# Autodesk Inventor assembly: OttosBreadboard_ASM
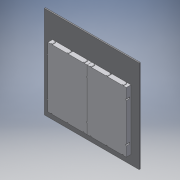
[picture p0: Inventor's stored thumbnail of the model, 180x180]
Saved by Autodesk Inventor 2016 (Build 200138000, 138)
## iProperties
Created: 2018-06-19
Part Number: OttosBreadboard_ASM
Document SubType Name: Assembly
Designer: suku
Author: suku
## Documents named in this file (3)
- I:\SukuWc\Otto's DIY\Core\Breadboard\OttosBreadboard_ASM.iam
- I:\SukuWc\Otto's DIY\Core\Breadboard\OttosBreadboard.ipt
- I:\SukuWc\Otto's DIY\Core\Breadboard\Frontpanel.ipt
## Components (3 placed, 2 different names)
1. OttosBreadboard:1 — Flush:1, Flush:2, Mate:1
2. OttosBreadboard:2 — Flush:1, Flush:2, Mate:1, Flush:3
3. Frontpanel:1 — Flush:3
## Relationships (4: Flush 3, Mate 1)
- Flush:1: OttosBreadboard:1 ↔ OttosBreadboard:2
- Flush:2: OttosBreadboard:1 ↔ OttosBreadboard:2
- Mate:1: OttosBreadboard:1 ↔ OttosBreadboard:2
- Flush:3: OttosBreadboard:2 ↔ Frontpanel:1
